# Autodesk Inventor assembly: 217-2778-001 Rev2_NCQ8A075-050M
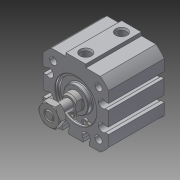
[picture p0: Inventor's stored thumbnail of the model, 180x180]
Saved by Autodesk Inventor 2014 SP1 (Build 180222100, 222)
## iProperties
Created: 2014-01-07
Part Number: 217-2778-001 Rev2_NCQ8A075-050M
Document SubType Name: Assembly
Designer: Andrew Toennies
Mass: 69.0266 g
Surface Area: 118.03 cm^2
Volume: 20.0572 cm^3
Density: 3.44149 g/cm^3
Author: Andrew Toennies
## Documents named in this file (5)
- C:\Users\Moses\Documents\GitHub\2014buildCAD\Shooter\Constrained 2 Speed Ball Shifter\217-2778-001 Rev2_NCQ8A075-050M.iam
- C:\Users\Moses\Documents\GitHub\2014buildCAD\Shooter\Constrained 2 Speed Ball Shifter\217-2778-NCQ8A075-050M_NCQ8 Tube_075A.ipt
- C:\Users\Moses\Documents\GitHub\2014buildCAD\Shooter\Constrained 2 Speed Ball Shifter\217-2778-NCQ8A075-050M_NCQ8 Rod_075M.ipt
- C:\Users\Moses\Documents\GitHub\2014buildCAD\Shooter\Constrained 2 Speed Ball Shifter\217-2778-NCQ8A075-050M_Snap Ring_075.ipt
- C:\Users\Moses\Documents\GitHub\2014buildCAD\Shooter\Constrained 2 Speed Ball Shifter\217-2778-NCQ8A075-050M_1032_Nut_90545A111.ipt
## Components (4 placed, 4 different names)
1. 217-2778-NCQ8A075-050M_NCQ8 Tube_075A_77 — Mate:1
2. 217-2778-NCQ8A075-050M_NCQ8 Rod_075M_78 — Mate:1
3. 217-2778-NCQ8A075-050M_Snap Ring_075_79
4. 217-2778-NCQ8A075-050M_1032_Nut_90545A111_80
## Relationships (1: Mate 1)
- Mate:1: 217-2778-NCQ8A075-050M_NCQ8 Tube_075A_77 ↔ 217-2778-NCQ8A075-050M_NCQ8 Rod_075M_78
